# Autodesk Inventor assembly: elbow_1
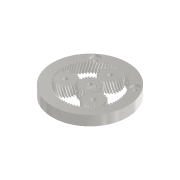
[picture p0: Inventor's stored thumbnail of the model, 180x180]
Saved by Autodesk Inventor 2020.2 (Build 242310000, 310)
## iProperties
Created: 2020-04-12
Part Number: elbow_1
Document SubType Name: Assembly
Designer: Bardo91
Author: Bardo91
## Documents named in this file (4)
- D:\programming\bioarm\hardware\2. arm\elbow_1.iam
- D:\programming\bioarm\hardware\2. arm\elbow_gear_ext.ipt
- D:\programming\bioarm\hardware\2. arm\elbow_gear_int_1.ipt
- D:\programming\bioarm\hardware\2. arm\elbow_gear_int_1_MIR.ipt
## Components (5 placed, 3 different names)
1. Spur Gear2:2
2. Spur Gear1:1
3. Spur Gear1:2
4. Spur Gear1:3
5. elbow_gear_int_1_MIR:1
## Relationships (10: Mate 6, Flush 4)
- [Flush]: Spur Gear2:2 ↔ Spur Gear1:2
- [Flush]: Spur Gear2:2 ↔ Spur Gear1:1
- [Flush]: Spur Gear2:2 ↔ Spur Gear1:3
- [Mate]: Spur Gear2:2 ↔ elbow_gear_int_1_MIR:1
- [Mate] (15 mm): Spur Gear1:3 ↔ elbow_gear_int_1_MIR:1
- [Mate] (15 mm): Spur Gear1:1 ↔ elbow_gear_int_1_MIR:1
- [Mate] (15 mm): Spur Gear1:2 ↔ elbow_gear_int_1_MIR:1
- [Flush]: Spur Gear1:1 ↔ elbow_gear_int_1_MIR:1
- [Mate] (26 mm): Spur Gear1:1 ↔ Spur Gear1:2
- [Mate] (26 mm): Spur Gear1:2 ↔ Spur Gear1:3
